# Autodesk Inventor assembly: Cim and p80 rough
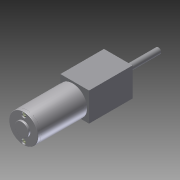
[picture p0: Inventor's stored thumbnail of the model, 180x180]
Saved by Autodesk Inventor 2013 (Build 170138000, 138)
## iProperties
Created: 2013-02-03
Part Number: Cim and p80 rough
Document SubType Name: Assembly
Designer: Arpan
Mass: 755.448 g
Surface Area: 766.246 cm^2
Volume: 755.448 cm^3
Density: 1 g/cm^3
Author: Arpan
## Documents named in this file (3)
- C:\Users\Moses\Documents\GitHub\frc2013CAD\Cimber actual\Cim and p80 rough.iam
- C:\Users\Moses\Documents\GitHub\frc2013CAD\Cimber actual\p80 space thing.ipt
- C:\Users\Moses\Documents\GitHub\frc2013CAD\Cimber actual\Imported Components\CIM Motor\CIM Motor.iam
## Components (2 placed, 2 different names)
1. p80 space thing:1 — Mate:1, Mate:2
2. CIM Motor:1 [sub-assembly] — Mate:1, Mate:2
## Relationships (2: Mate 2)
- Mate:1: p80 space thing:1 ↔ CIM Motor:1
- Mate:2: p80 space thing:1 ↔ CIM Motor:1
